# Autodesk Inventor assembly: __VK_WT
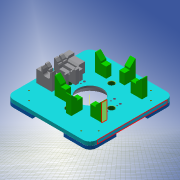
[picture p0: Inventor's stored thumbnail of the model, 180x180]
Saved by Autodesk Inventor 2019 (Build 230136000, 136)
## iProperties
Created: 2023-11-19
Part Number: __VK_WT
Material: Generisch
Document SubType Name: Assembly
Designer: RP
Author: RP
## Documents named in this file (9)
- C:\Users\RP\Documents\Inventor\___Projekt_Useless_Box\_Verkettung\__VK_WT.iam
- C:\Users\RP\Documents\Inventor\___Projekt_Useless_Box\_Verkettung\__VK_Werkstückträger_240.ipt
- C:\Users\RP\Documents\Inventor\___Projekt_Useless_Box\_Verkettung\_WT_Aufnahme1.ipt
- C:\Users\RP\Documents\Inventor\___Projekt_Useless_Box\_Verkettung\_WT_Aufnahme_Antriebseinheit1.ipt
- C:\Users\RP\Documents\Inventor\___Projekt_Useless_Box\_Verkettung\_WT_Aufnahme_Antriebseinheit2.ipt
- C:\Users\RP\Documents\Inventor\___Projekt_Useless_Box\_Verkettung\_WT_Aufnahme_Antriebseinheit3.ipt
- C:\Users\RP\Documents\Inventor\___Projekt_Useless_Box\_Verkettung\_WT_Aufnahme_Antriebseinheit4.ipt
- C:\Users\RP\Documents\Inventor\___Projekt_Useless_Box\_Verkettung\_WT_Aufnahme_Antriebseinheit5.ipt
- C:\Users\RP\Documents\Inventor\___Projekt_Useless_Box\_Verkettung\_WT_Aufnahme_Antriebseinheit6.ipt
## Components (14 placed, 8 different names)
1. __VK_Werkstückträger_240:1 — Fluchtend:4, Fluchtend:5, Fluchtend:6, Fluchtend:7, Fluchtend:10, Fluchtend:11, Fluchtend:12
2. _WT_Aufnahme_Antriebseinheit5:1 — Passend:16, Fluchtend:23
3. _WT_Aufnahme_Antriebseinheit3:1 — Passend:15
4. _WT_Aufnahme_Antriebseinheit4:1 — Passend:15
5. _WT_Aufnahme_Antriebseinheit6:1 — Passend:16, Passend:17
6. _WT_Aufnahme_Antriebseinheit2:1 — Passend:17
7. _WT_Aufnahme_Antriebseinheit1:1 — Fluchtend:23
8. _WT_Aufnahme_Antriebseinheit1:2
9. _WT_Aufnahme1:2 — Fluchtend:4
10. _WT_Aufnahme1:3 — Fluchtend:6, Fluchtend:12
11. _WT_Aufnahme1:4 — Fluchtend:9, Fluchtend:11
12. _WT_Aufnahme1:1 — Fluchtend:5, Fluchtend:9, Fluchtend:10
13. _WT_Aufnahme1:5 — Fluchtend:8
14. _WT_Aufnahme1:6 — Fluchtend:7, Fluchtend:8
## Relationships (39: Flush 22, Mate 17)
- [Mate]: __VK_Werkstückträger_240:1 ↔ _WT_Aufnahme1:3
- [Mate]: __VK_Werkstückträger_240:1 ↔ _WT_Aufnahme1:2
- [Mate]: __VK_Werkstückträger_240:1 ↔ _WT_Aufnahme1:4
- [Mate]: __VK_Werkstückträger_240:1 ↔ _WT_Aufnahme1:1
- [Mate]: __VK_Werkstückträger_240:1 ↔ _WT_Aufnahme1:5
- [Flush]: _WT_Aufnahme1:2 ↔ _WT_Aufnahme1:3
- [Mate]: __VK_Werkstückträger_240:1 ↔ _WT_Aufnahme1:6
- [Flush]: _WT_Aufnahme1:1 ↔ _WT_Aufnahme1:5
- [Flush]: _WT_Aufnahme1:4 ↔ _WT_Aufnahme1:6
- Fluchtend:4 [Flush] (12.8 mm): __VK_Werkstückträger_240:1 ↔ _WT_Aufnahme1:2
- Fluchtend:5 [Flush] (69 mm): __VK_Werkstückträger_240:1 ↔ _WT_Aufnahme1:1
- Fluchtend:6 [Flush] (42.2 mm): __VK_Werkstückträger_240:1 ↔ _WT_Aufnahme1:3
- Fluchtend:7 [Flush] (-36 mm): __VK_Werkstückträger_240:1 ↔ _WT_Aufnahme1:6
- Fluchtend:8 [Flush]: _WT_Aufnahme1:5 ↔ _WT_Aufnahme1:6
- Fluchtend:9 [Flush]: _WT_Aufnahme1:4 ↔ _WT_Aufnahme1:1
- Fluchtend:10 [Flush] (39.8 mm): __VK_Werkstückträger_240:1 ↔ _WT_Aufnahme1:1
- Fluchtend:11 [Flush] (69.2 mm): __VK_Werkstückträger_240:1 ↔ _WT_Aufnahme1:4
- Fluchtend:12 [Flush] (-128.5 mm): __VK_Werkstückträger_240:1 ↔ _WT_Aufnahme1:3
- [Flush]: _WT_Aufnahme_Antriebseinheit5:1 ↔ _WT_Aufnahme_Antriebseinheit3:1
- [Flush]: _WT_Aufnahme_Antriebseinheit5:1 ↔ _WT_Aufnahme_Antriebseinheit3:1
- [Mate]: __VK_Werkstückträger_240:1 ↔ _WT_Aufnahme_Antriebseinheit5:1
- [Flush]: _WT_Aufnahme_Antriebseinheit5:1 ↔ _WT_Aufnahme_Antriebseinheit4:1
- [Flush]: _WT_Aufnahme_Antriebseinheit5:1 ↔ _WT_Aufnahme_Antriebseinheit4:1
- [Mate]: __VK_Werkstückträger_240:1 ↔ _WT_Aufnahme_Antriebseinheit6:1
- [Mate]: __VK_Werkstückträger_240:1 ↔ _WT_Aufnahme_Antriebseinheit2:1
- [Flush]: _WT_Aufnahme_Antriebseinheit6:1 ↔ _WT_Aufnahme_Antriebseinheit2:1
- [Mate]: __VK_Werkstückträger_240:1 ↔ _WT_Aufnahme_Antriebseinheit1:1
- [Mate]: _WT_Aufnahme_Antriebseinheit6:1 ↔ _WT_Aufnahme_Antriebseinheit1:1
- [Mate]: __VK_Werkstückträger_240:1 ↔ _WT_Aufnahme_Antriebseinheit1:2
- [Mate]: _WT_Aufnahme_Antriebseinheit2:1 ↔ _WT_Aufnahme_Antriebseinheit1:2
- [Flush]: _WT_Aufnahme_Antriebseinheit6:1 ↔ _WT_Aufnahme_Antriebseinheit1:1
- [Flush] (12 mm): __VK_Werkstückträger_240:1 ↔ _WT_Aufnahme_Antriebseinheit1:1
- [Flush]: _WT_Aufnahme_Antriebseinheit2:1 ↔ _WT_Aufnahme_Antriebseinheit1:2
- [Mate]: _WT_Aufnahme_Antriebseinheit3:1 ↔ _WT_Aufnahme_Antriebseinheit1:2
- [Flush] (31.9 mm): _WT_Aufnahme_Antriebseinheit6:1 ↔ _WT_Aufnahme1:3
- Passend:15 [Mate] (4 mm): _WT_Aufnahme_Antriebseinheit3:1 ↔ _WT_Aufnahme_Antriebseinheit4:1
- Passend:16 [Mate] (3 mm): _WT_Aufnahme_Antriebseinheit5:1 ↔ _WT_Aufnahme_Antriebseinheit6:1
- Passend:17 [Mate] (53.2 mm): _WT_Aufnahme_Antriebseinheit6:1 ↔ _WT_Aufnahme_Antriebseinheit2:1
- Fluchtend:23 [Flush]: _WT_Aufnahme_Antriebseinheit5:1 ↔ _WT_Aufnahme_Antriebseinheit1:1
## Named parameters: d179_d52 = 0 mm, d180_d53 = 12 mm
